# Autodesk Inventor assembly: deltaRobot
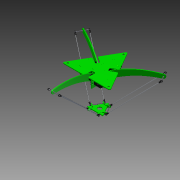
[picture p0: Inventor's stored thumbnail of the model, 180x180]
Saved by Autodesk Inventor 2012 (Build 160160000, 160)
## iProperties
Created: 2013-10-01
Part Number: deltaRobot
Document SubType Name: Assembly
Designer: Nick
Author: Nick
## Documents named in this file (10)
- C:\Users\Nick\Documents\GitHub\DeltaRobot\cad_v1\deltaRobot.iam
- C:\Users\Nick\Documents\GitHub\DeltaRobot\cad_v1\brazo.ipt
- C:\Users\Nick\Documents\GitHub\DeltaRobot\cad_v1\Imported Components\PowerHD1501MG_STEP\PowerHD1501MG_STEP.ipt
- C:\Users\Nick\Documents\GitHub\DeltaRobot\cad_v1\base.ipt
- C:\Users\Nick\Documents\GitHub\DeltaRobot\cad_v1\actuator.ipt
- C:\Users\Nick\Documents\GitHub\DeltaRobot\cad_v1\top_holder.ipt
- C:\Users\Nick\Documents\GitHub\DeltaRobot\cad_v1\rod_assembly.iam
- C:\Users\Nick\Documents\GitHub\DeltaRobot\cad_v1\servo_holder.ipt
- C:\Users\Nick\Documents\GitHub\DeltaRobot\cad_v1\servo_holer2.ipt
- C:\Users\Nick\Documents\GitHub\DeltaRobot\cad_v1\servo_holder3.ipt
## Components (26 placed, 9 different names)
1. base:1 — Mate:61, Mate:62, Mate:63, Mate:73, Mate:74, Mate:75, Mate:76, Mate:77, Mate:78, Mate:88, Mate:89, Mate:90, Mate:91, Mate:92, Mate:93, Mate:94, Mate:95, Mate:96
2. brazo:2 — Mate:1, Mate:5, Mate:58, Mate:59
3. brazo:3 — Mate:3, Mate:6, Mate:60
4. PowerHD1501MG_STEP:1 — Mate:1, Mate:5, Mate:62, Mate:67, Mate:68, Mate:69, Mate:85
5. PowerHD1501MG_STEP:2 — Mate:54, Mate:55, Mate:61, Mate:70, Mate:71, Mate:72, Mate:82
6. PowerHD1501MG_STEP:3 — Mate:3, Mate:6, Mate:63, Mate:64, Mate:65, Mate:66
7. actuator:1 — Mate:29, Mate:30, Mate:31, Mate:32, Mate:33, Mate:34, Mate:36, Mate:37, Mate:38, Mate:39, Mate:40, Mate:41, Mate:42, Mate:43, Mate:44, Mate:45, Mate:46, Mate:47
8. top_holder:1 — Mate:29, Mate:30, Mate:31
9. top_holder:2 — Mate:32, Mate:33, Mate:34, Mate:50, Mate:51
10. top_holder:3 — Mate:36, Mate:40, Mate:41, Mate:49
11. top_holder:4 — Mate:37, Mate:42, Mate:43, Mate:48
12. top_holder:5 — Mate:38, Mate:45, Mate:47
13. top_holder:6 — Mate:39, Mate:44, Mate:46, Mate:52, Mate:53
14. rod_assembly:1 [sub-assembly] — Mate:52, Mate:53, Mate:56, Mate:57
15. rod_assembly:2 [sub-assembly] — Mate:50, Mate:51, Mate:60
16. rod_assembly:3 [sub-assembly] — Mate:48, Mate:49, Mate:58, Mate:59
17. brazo:4 — Mate:54, Mate:55, Mate:56, Mate:57
18. servo_holder:1 — Mate:70, Mate:71, Mate:72, Mate:75, Mate:76, Mate:83, Mate:84
19. servo_holder:2 — Mate:67, Mate:68, Mate:69, Mate:77, Mate:78, Mate:86, Mate:87
20. servo_holder:3 — Mate:64, Mate:65, Mate:66, Mate:73, Mate:74, Mate:79, Mate:80, Mate:81
21. servo_holer2:1 — Mate:85, Mate:86, Mate:87
22. servo_holer2:2 — Mate:82, Mate:83, Mate:84
23. servo_holer2:3 — Mate:79, Mate:80, Mate:81
24. servo_holder3:1 — Mate:90, Mate:91, Mate:92
25. servo_holder3:2 — Mate:88, Mate:93, Mate:94
26. servo_holder3:3 — Mate:89, Mate:95, Mate:96
## Relationships (71: Mate 71)
- Mate:1: brazo:2 ↔ PowerHD1501MG_STEP:1
- Mate:3: brazo:3 ↔ PowerHD1501MG_STEP:3
- Mate:5: brazo:2 ↔ PowerHD1501MG_STEP:1
- Mate:6: brazo:3 ↔ PowerHD1501MG_STEP:3
- Mate:29: actuator:1 ↔ top_holder:1
- Mate:30: actuator:1 ↔ top_holder:1
- Mate:31: actuator:1 ↔ top_holder:1
- Mate:32: actuator:1 ↔ top_holder:2
- Mate:33: actuator:1 ↔ top_holder:2
- Mate:34: actuator:1 ↔ top_holder:2
- Mate:36: actuator:1 ↔ top_holder:3
- Mate:37: actuator:1 ↔ top_holder:4
- Mate:38: actuator:1 ↔ top_holder:5
- Mate:39: actuator:1 ↔ top_holder:6
- Mate:40: actuator:1 ↔ top_holder:3
- Mate:41: actuator:1 ↔ top_holder:3
- Mate:42: actuator:1 ↔ top_holder:4
- Mate:43: actuator:1 ↔ top_holder:4
- Mate:44: actuator:1 ↔ top_holder:6
- Mate:45: actuator:1 ↔ top_holder:5
- Mate:46: actuator:1 ↔ top_holder:6
- Mate:47: actuator:1 ↔ top_holder:5
- Mate:48: top_holder:4 ↔ rod_assembly:3
- Mate:49: top_holder:3 ↔ rod_assembly:3
- Mate:50: top_holder:2 ↔ rod_assembly:2
- Mate:51: top_holder:2 ↔ rod_assembly:2
- Mate:52: top_holder:6 ↔ rod_assembly:1
- Mate:53: top_holder:6 ↔ rod_assembly:1
- Mate:54: PowerHD1501MG_STEP:2 ↔ brazo:4
- Mate:55: PowerHD1501MG_STEP:2 ↔ brazo:4
- Mate:56: rod_assembly:1 ↔ brazo:4
- Mate:57 (1.5 mm): rod_assembly:1 ↔ brazo:4
- Mate:58: brazo:2 ↔ rod_assembly:3
- Mate:59 (-1.5 mm): brazo:2 ↔ rod_assembly:3
- Mate:60: brazo:3 ↔ rod_assembly:2
- Mate:61: base:1 ↔ PowerHD1501MG_STEP:2
- Mate:62: base:1 ↔ PowerHD1501MG_STEP:1
- Mate:63: base:1 ↔ PowerHD1501MG_STEP:3
- Mate:64: PowerHD1501MG_STEP:3 ↔ servo_holder:3
- Mate:65: PowerHD1501MG_STEP:3 ↔ servo_holder:3
- Mate:66: PowerHD1501MG_STEP:3 ↔ servo_holder:3
- Mate:67: PowerHD1501MG_STEP:1 ↔ servo_holder:2
- Mate:68: PowerHD1501MG_STEP:1 ↔ servo_holder:2
- Mate:69: PowerHD1501MG_STEP:1 ↔ servo_holder:2
- Mate:70: PowerHD1501MG_STEP:2 ↔ servo_holder:1
- Mate:71: PowerHD1501MG_STEP:2 ↔ servo_holder:1
- Mate:72: PowerHD1501MG_STEP:2 ↔ servo_holder:1
- Mate:73: base:1 ↔ servo_holder:3
- Mate:74: base:1 ↔ servo_holder:3
- Mate:75: base:1 ↔ servo_holder:1
- Mate:76: base:1 ↔ servo_holder:1
- Mate:77: base:1 ↔ servo_holder:2
- Mate:78: base:1 ↔ servo_holder:2
- Mate:79: servo_holder:3 ↔ servo_holer2:3
- Mate:80: servo_holder:3 ↔ servo_holer2:3
- Mate:81: servo_holder:3 ↔ servo_holer2:3
- Mate:82: PowerHD1501MG_STEP:2 ↔ servo_holer2:2
- Mate:83: servo_holder:1 ↔ servo_holer2:2
- Mate:84: servo_holder:1 ↔ servo_holer2:2
- Mate:85: PowerHD1501MG_STEP:1 ↔ servo_holer2:1
- Mate:86: servo_holder:2 ↔ servo_holer2:1
- Mate:87: servo_holder:2 ↔ servo_holer2:1
- Mate:88: base:1 ↔ servo_holder3:2
- Mate:89: base:1 ↔ servo_holder3:3
- Mate:90: base:1 ↔ servo_holder3:1
- Mate:91: base:1 ↔ servo_holder3:1
- Mate:92: base:1 ↔ servo_holder3:1
- Mate:93: base:1 ↔ servo_holder3:2
- Mate:94: base:1 ↔ servo_holder3:2
- Mate:95: base:1 ↔ servo_holder3:3
- Mate:96: base:1 ↔ servo_holder3:3
